# Autodesk Inventor assembly: thicc
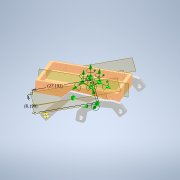
[picture p0: Inventor's stored thumbnail of the model, 180x180]
Saved by Autodesk Inventor 2020 (Build 240168000, 168)
## iProperties
Created: 2020-08-04
Part Number: thicc
Document SubType Name: Assembly
Designer: Manish
Author: Manish
## Documents named in this file (6)
- C:\Users\Manish\Documents\inventor\thicc.iam
- C:\Users\Manish\Documents\inventor\Ref\basefresh.ipt
- C:\Users\Public\Documents\Autodesk\Inventor 2020\bogie1.ipt
- C:\Users\Public\Documents\Autodesk\Inventor 2020\bogie2.ipt
- C:\Users\Public\Documents\Autodesk\Inventor 2020\bogie1_MIR.ipt
- C:\Users\Public\Documents\Autodesk\Inventor 2020\bogie2_MIR.ipt
## Components (5 placed, 5 different names)
1. basefresh:1 — Flush:1, Flush:2, Rotation:1, Rotation:2, Rotational:1
2. bogie1:1 — Flush:1, Flush:2, Rotation:1, Flush:3, Flush:5, Rotation:2, Rotation:3, Rotational:1, Rotational:2
3. bogie2:1 — Flush:3, Flush:5, Rotation:3, Rotational:2
4. bogie1_MIR:1 — Rotation:4, Mate:1, Mate:2, Rotational:3
5. bogie2_MIR:1 — Rotation:4, Mate:1, Mate:2, Rotational:3
## Relationships (13: Flush 4, RelateRotation 4, RevoluteJoint 3, Mate 2)
- Flush:1: basefresh:1 ↔ bogie1:1
- Flush:2: basefresh:1 ↔ bogie1:1
- Rotation:1 [RelateRotation] (1 ul): basefresh:1 ↔ bogie1:1
- Flush:3: bogie1:1 ↔ bogie2:1
- Flush:5: bogie1:1 ↔ bogie2:1
- Rotation:2 [RelateRotation] (1 ul): basefresh:1 ↔ bogie1:1
- Rotation:3 [RelateRotation] (1 ul): bogie1:1 ↔ bogie2:1
- Rotational:1 [RevoluteJoint]: basefresh:1 ↔ bogie1:1
- Rotational:2 [RevoluteJoint]: bogie1:1 ↔ bogie2:1
- Rotation:4 [RelateRotation] (1 ul): bogie1_MIR:1 ↔ bogie2_MIR:1
- Mate:1: bogie1_MIR:1 ↔ bogie2_MIR:1
- Mate:2: bogie1_MIR:1 ↔ bogie2_MIR:1
- Rotational:3 [RevoluteJoint]: bogie1_MIR:1 ↔ bogie2_MIR:1
